# Autodesk Inventor assembly: ArkFullTest
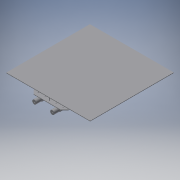
[picture p0: Inventor's stored thumbnail of the model, 180x180]
Saved by Autodesk Inventor 2018 (Build 220112000, 112)
## iProperties
Created: 2019-11-10
Part Number: ArkFullTest
Material: Типовые
Document SubType Name: Assembly
Designer: cosko
Author: cosko
## Documents named in this file (17)
- C:\Users\cosko\source\repos\Arkanoid-robot\Ark.ipt\Kick 25-370\ArkFullTest.iam
- C:\Users\cosko\source\repos\Arkanoid-robot\Ark.ipt\Up base.ipt
- C:\Users\cosko\source\repos\Arkanoid-robot\Ark.ipt\Motor.ipt
- C:\Users\cosko\source\repos\Arkanoid-robot\Ark.ipt\sleeve.ipt
- C:\Users\cosko\source\repos\Arkanoid-robot\Ark.ipt\Wheel.ipt
- C:\Users\cosko\source\repos\Arkanoid-robot\Ark.ipt\Mount for motor.ipt
- C:\Users\cosko\source\repos\Arkanoid-robot\Ark.ipt\FailVersions\Stick.ipt
- C:\Users\cosko\source\repos\Arkanoid-robot\Ark.ipt\Side control right.ipt
- C:\Users\cosko\source\repos\Arkanoid-robot\Ark.ipt\Side control left.ipt
- C:\Users\cosko\source\repos\Arkanoid-robot\Ark.ipt\Screw.ipt
- C:\Users\cosko\source\repos\Arkanoid-robot\Ather\ipt\Arduino\Arduino Nano.ipt
- C:\Users\cosko\source\repos\Arkanoid-robot\Ark.ipt\Floor.ipt
- C:\Users\cosko\source\repos\Arkanoid-robot\Ark.ipt\Kick male.ipt
- C:\Users\cosko\source\repos\Arkanoid-robot\Ark.ipt\Kick female.ipt
- C:\Users\cosko\source\repos\Arkanoid-robot\Ark.ipt\Shoulder .ipt
- C:\Users\cosko\source\repos\Arkanoid-robot\Ark.ipt\sleeve for kick.ipt
- C:\Users\cosko\source\repos\Arkanoid-robot\Ark.ipt\Kick 25-370\Ark.ipt\Down base.ipt
## Components (26 placed, 16 different names)
1. Up base:1 — Совмещение:3, Совмещение:4, Заподлицо:3, Заподлицо:4, Заподлицо:5, Заподлицо:9, Совмещение:6, Совмещение:7, Совмещение:11, Совмещение:13, Вставка:13, Вставка:14, Вставка:15, Совмещение:14, Совмещение:21, Заподлицо:17, Заподлицо:18, Вставка:26, Вставка:27, Вставка:28, Вставка:29
2. Motor:1 — Совмещение:1, Касательность:1, Вставка:1, Заподлицо:2
3. sleeve:1 — Вставка:1, Вставка:2, Вставка:3
4. Wheel:1 — Вставка:2, Вставка:3, Касательность:3, Заподлицо:8
5. Mount for motor:1 — Совмещение:1, Касательность:1, Совмещение:4, Заподлицо:1, Заподлицо:5, Вставка:26, Вставка:27
6. Motor:2 — Совмещение:2, Касательность:2, Вставка:4, Заподлицо:2
7. Mount for motor:2 — Совмещение:2, Касательность:2, Совмещение:3, Заподлицо:1, Заподлицо:3, Заподлицо:4, Совмещение:15, Заподлицо:14, Вставка:28, Вставка:29
8. sleeve:2 — Вставка:4, Вставка:5, Вставка:6
9. Wheel:2 — Вставка:5, Вставка:6, Касательность:4
10. Stick:1 — Касательность:3, Касательность:4, Заподлицо:8, Заподлицо:9, Совмещение:8, Совмещение:9, Совмещение:10, Совмещение:12, Совмещение:18
11. Side control right:1 — Заподлицо:10, Совмещение:6, Совмещение:7, Совмещение:8, Заподлицо:11
12. Side control left:1 — Заподлицо:10, Совмещение:9, Заподлицо:11
13. Side control right:2 — Заподлицо:12, Заподлицо:13, Совмещение:10, Совмещение:11, Совмещение:13
14. Side control left:2 — Заподлицо:12, Заподлицо:13, Совмещение:12
15. Screw:1 — Вставка:13, Вставка:31
16. Screw:2 — Вставка:14, Вставка:30
17. Screw:3 — Вставка:15
18. Arduino Nano:1 — Совмещение:14, Совмещение:15, Заподлицо:14
19. Floor:1 — Совмещение:18
20. Kick male:1 — Совмещение:19, Совмещение:20, Заподлицо:15, Заподлицо:16, Вставка:21, Вставка:22
21. Kick female:1 — Совмещение:19, Совмещение:20, Заподлицо:15, Заподлицо:16
22. Motor:3 — Вставка:19, Вставка:23
23. Mount for motor:3 — Вставка:19, Совмещение:21, Заподлицо:17, Заподлицо:18
24. Shoulder :1 — Вставка:21, Вставка:22, Вставка:24, Вставка:25
25. sleeve for kick:1 — Вставка:23, Вставка:24, Вставка:25
26. Down base:2 — Вставка:30, Вставка:31
## Relationships (59: Insert 21, Mate 18, Flush 16, Tangent 4)
- Совмещение:1 [Mate]: Motor:1 ↔ Mount for motor:1
- Касательность:1 [Tangent]: Motor:1 ↔ Mount for motor:1
- Совмещение:2 [Mate]: Motor:2 ↔ Mount for motor:2
- Касательность:2 [Tangent]: Motor:2 ↔ Mount for motor:2
- Вставка:1 [Insert]: Motor:1 ↔ sleeve:1
- Вставка:2 [Insert]: sleeve:1 ↔ Wheel:1
- Вставка:3 [Insert]: sleeve:1 ↔ Wheel:1
- Вставка:4 [Insert]: Motor:2 ↔ sleeve:2
- Вставка:5 [Insert]: sleeve:2 ↔ Wheel:2
- Вставка:6 [Insert]: sleeve:2 ↔ Wheel:2
- Совмещение:3 [Mate]: Up base:1 ↔ Mount for motor:2
- Совмещение:4 [Mate]: Up base:1 ↔ Mount for motor:1
- Заподлицо:1 [Flush]: Mount for motor:1 ↔ Mount for motor:2
- Заподлицо:2 [Flush]: Motor:1 ↔ Motor:2
- Заподлицо:3 [Flush] (10 mm): Up base:1 ↔ Mount for motor:2
- Заподлицо:4 [Flush] (20 mm): Up base:1 ↔ Mount for motor:2
- Заподлицо:5 [Flush] (20 mm): Up base:1 ↔ Mount for motor:1
- Касательность:3 [Tangent]: Wheel:1 ↔ Stick:1
- Касательность:4 [Tangent]: Wheel:2 ↔ Stick:1
- Заподлицо:8 [Flush] (2.5 mm): Wheel:1 ↔ Stick:1
- Заподлицо:9 [Flush]: Up base:1 ↔ Stick:1
- Заподлицо:10 [Flush]: Side control right:1 ↔ Side control left:1
- Совмещение:6 [Mate]: Up base:1 ↔ Side control right:1
- Совмещение:7 [Mate]: Up base:1 ↔ Side control right:1
- Совмещение:8 [Mate]: Stick:1 ↔ Side control right:1
- Совмещение:9 [Mate]: Stick:1 ↔ Side control left:1
- Заподлицо:11 [Flush]: Side control right:1 ↔ Side control left:1
- Заподлицо:12 [Flush]: Side control right:2 ↔ Side control left:2
- Заподлицо:13 [Flush]: Side control right:2 ↔ Side control left:2
- Совмещение:10 [Mate]: Stick:1 ↔ Side control right:2
- Совмещение:11 [Mate]: Up base:1 ↔ Side control right:2
- Совмещение:12 [Mate]: Stick:1 ↔ Side control left:2
- Совмещение:13 [Mate]: Up base:1 ↔ Side control right:2
- Вставка:13 [Insert]: Up base:1 ↔ Screw:1
- Вставка:14 [Insert]: Up base:1 ↔ Screw:2
- Вставка:15 [Insert]: Up base:1 ↔ Screw:3
- Совмещение:14 [Mate]: Up base:1 ↔ Arduino Nano:1
- Совмещение:15 [Mate]: Mount for motor:2 ↔ Arduino Nano:1
- Заподлицо:14 [Flush]: Mount for motor:2 ↔ Arduino Nano:1
- Совмещение:18 [Mate] (100 mm): Stick:1 ↔ Floor:1
- Совмещение:19 [Mate]: Kick male:1 ↔ Kick female:1
- Совмещение:20 [Mate]: Kick male:1 ↔ Kick female:1
- Заподлицо:15 [Flush]: Kick male:1 ↔ Kick female:1
- Заподлицо:16 [Flush]: Kick male:1 ↔ Kick female:1
- Вставка:19 [Insert]: Motor:3 ↔ Mount for motor:3
- Совмещение:21 [Mate]: Up base:1 ↔ Mount for motor:3
- Заподлицо:17 [Flush]: Up base:1 ↔ Mount for motor:3
- Заподлицо:18 [Flush]: Up base:1 ↔ Mount for motor:3
- Вставка:21 [Insert]: Kick male:1 ↔ Shoulder :1
- Вставка:22 [Insert]: Kick male:1 ↔ Shoulder :1
- Вставка:23 [Insert]: Motor:3 ↔ sleeve for kick:1
- Вставка:24 [Insert]: Shoulder :1 ↔ sleeve for kick:1
- Вставка:25 [Insert]: Shoulder :1 ↔ sleeve for kick:1
- Вставка:26 [Insert]: Up base:1 ↔ Mount for motor:1
- Вставка:27 [Insert]: Up base:1 ↔ Mount for motor:1
- Вставка:28 [Insert]: Up base:1 ↔ Mount for motor:2
- Вставка:29 [Insert]: Up base:1 ↔ Mount for motor:2
- Вставка:30 [Insert]: Screw:2 ↔ Down base:2
- Вставка:31 [Insert]: Screw:1 ↔ Down base:2
